# Autodesk Inventor assembly: 2024-220-Hard-Stop
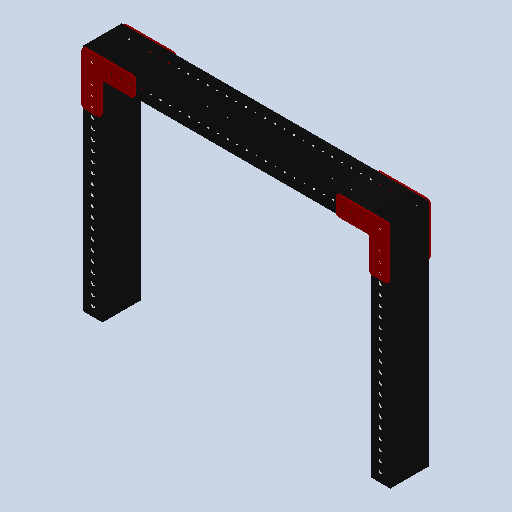
[picture p0: Inventor's stored thumbnail of the model, 512x512]
Saved by Autodesk Inventor 2024 (Build 280153000, 153)
## iProperties
Created: 2024-01-23
Part Number: 2024-220-Hard-Stop
Document SubType Name: Assembly
Designer: rohan
Author: rohan
## Documents named in this file (5)
- C:\Users\5652160\OneDrive - Hillsborough County Public Schools\Robotics\FIRST-Robotics-Competition\Crescendo\Minotaur-Crescendo-Robot\Structure\Superstructure\Angle-Shootaur\2024-220-Hard-Stop.iam
- C:\Users\5652160\OneDrive - Hillsborough County Public Schools\Robotics\FIRST-Robotics-Competition\Crescendo\Minotaur-Crescendo-Robot\Structure\Superstructure\Angle-Shootaur\2024-220-001-Right-Stop-Support.ipt
- C:\Users\5652160\OneDrive - Hillsborough County Public Schools\Robotics\FIRST-Robotics-Competition\Crescendo\Minotaur-Crescendo-Robot\Structure\Superstructure\Angle-Shootaur\2024-220-003-Left-Stop-Support.ipt
- C:\Users\5652160\OneDrive - Hillsborough County Public Schools\Robotics\FIRST-Robotics-Competition\Crescendo\Minotaur-Crescendo-Robot\Structure\Superstructure\Angle-Shootaur\2024-220-002-Shootaur-Rest.ipt
- C:\Users\5652160\OneDrive - Hillsborough County Public Schools\Robotics\FIRST-Robotics-Competition\Crescendo\Minotaur-Crescendo-Robot\Structure\Gussets\THRIFYBOT-L-Gusset.ipt
## Components (7 placed, 4 different names)
1. 2024-220-001-Right-Stop-Support:1 — Mate:1, Flush:1, Flush:2, Mate:6, Flush:12
2. 2024-220-003-Left-Stop-Support:1 — Mate:2, Flush:3, Flush:4, Mate:5, Flush:10
3. 2024-220-002-Shootaur-Rest:1 — Mate:1, Flush:1, Flush:2, Mate:2, Flush:3, Flush:4, Flush:9, Flush:11
4. THRIFYBOT-L-Gusset:1 — Flush:5, Flush:6, Mate:3, Mate:6, Flush:11, Flush:12
5. THRIFYBOT-L-Gusset:2 — Flush:5, Flush:6, Mate:3
6. THRIFYBOT-L-Gusset:3 — Flush:7, Flush:8, Mate:4
7. THRIFYBOT-L-Gusset:4 — Flush:7, Flush:8, Mate:4, Mate:5, Flush:9, Flush:10
## Relationships (18: Flush 12, Mate 6)
- Mate:1: 2024-220-001-Right-Stop-Support:1 ↔ 2024-220-002-Shootaur-Rest:1
- Flush:1: 2024-220-001-Right-Stop-Support:1 ↔ 2024-220-002-Shootaur-Rest:1
- Flush:2: 2024-220-001-Right-Stop-Support:1 ↔ 2024-220-002-Shootaur-Rest:1
- Mate:2: 2024-220-003-Left-Stop-Support:1 ↔ 2024-220-002-Shootaur-Rest:1
- Flush:3: 2024-220-003-Left-Stop-Support:1 ↔ 2024-220-002-Shootaur-Rest:1
- Flush:4: 2024-220-003-Left-Stop-Support:1 ↔ 2024-220-002-Shootaur-Rest:1
- Flush:5: THRIFYBOT-L-Gusset:1 ↔ THRIFYBOT-L-Gusset:2
- Flush:6: THRIFYBOT-L-Gusset:1 ↔ THRIFYBOT-L-Gusset:2
- Mate:3 (50.8 mm): THRIFYBOT-L-Gusset:1 ↔ THRIFYBOT-L-Gusset:2
- Flush:7: THRIFYBOT-L-Gusset:3 ↔ THRIFYBOT-L-Gusset:4
- Flush:8: THRIFYBOT-L-Gusset:3 ↔ THRIFYBOT-L-Gusset:4
- Mate:4 (50.8 mm): THRIFYBOT-L-Gusset:3 ↔ THRIFYBOT-L-Gusset:4
- Mate:5: 2024-220-003-Left-Stop-Support:1 ↔ THRIFYBOT-L-Gusset:4
- Flush:9: 2024-220-002-Shootaur-Rest:1 ↔ THRIFYBOT-L-Gusset:4
- Flush:10: 2024-220-003-Left-Stop-Support:1 ↔ THRIFYBOT-L-Gusset:4
- Mate:6: 2024-220-001-Right-Stop-Support:1 ↔ THRIFYBOT-L-Gusset:1
- Flush:11: 2024-220-002-Shootaur-Rest:1 ↔ THRIFYBOT-L-Gusset:1
- Flush:12: 2024-220-001-Right-Stop-Support:1 ↔ THRIFYBOT-L-Gusset:1
